# Autodesk Inventor assembly: Jonathan's Printer
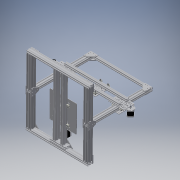
[picture p0: Inventor's stored thumbnail of the model, 180x180]
Saved by Autodesk Inventor 2016 (Build 200138000, 138)
## iProperties
Created: 2015-09-06
Part Number: Jonathan's Printer
Document SubType Name: Assembly
Designer: Solomon
Author: Solomon
## Documents named in this file (16)
- C:\Users\Solomon\Documents\Inventor\jonathan-printer\Jonathan's Printer.iam
- C:\Users\Solomon\Documents\Inventor\jonathan-printer\V Slot Part Files\Extrusions\vslot 20 x 40.ipt
- C:\Users\Solomon\Documents\Inventor\jonathan-printer\V Slot Part Files\Extrusions\vslot 20 x 20 v2.ipt
- C:\Users\Solomon\Documents\Inventor\jonathan-printer\V Slot Part Files\Brackets and Joining Plates\5 Hole 90 Degree Bracket.ipt
- C:\Users\Solomon\Documents\Inventor\jonathan-printer\V Slot Part Files\Extrusions\vslot 20 x 40 - 250mm.ipt
- C:\Users\Solomon\Documents\Inventor\jonathan-printer\V Slot Part Files\Brackets and Joining Plates\5 Hole T Joining Plate.ipt
- C:\Users\Solomon\Documents\Inventor\jonathan-printer\V Slot Part Files\Extrusions\vslot 20 x 40 - 125mm.ipt
- C:\Users\Solomon\Documents\Inventor\jonathan-printer\Z-axis Right.iam
- C:\Users\Solomon\Documents\Inventor\jonathan-printer\Z-axis Left Plate.iam
- C:\Users\Solomon\Documents\Inventor\jonathan-printer\X-carriage.iam
- C:\Users\Solomon\Documents\Inventor\jonathan-printer\y-carriage.iam
- C:\Users\Solomon\Documents\Inventor\jonathan-printer\M1173041- NEMA 17.ipt
- C:\Users\Solomon\Documents\Inventor\jonathan-printer\Imported Components\GT2_20tooth\GT2_20tooth.ipt
- C:\Users\Solomon\Documents\Inventor\jonathan-printer\V Slot Part Files\V Slot Plates\V-Slot Motor Mount Plate.ipt
- C:\Users\Solomon\Documents\Inventor\jonathan-printer\V Slot Part Files\V Slot Plates\VSlot Idler Pulley Plate.ipt
- C:\Users\Solomon\Documents\Inventor\jonathan-printer\V Slot Part Files\Pulleys Wheels Bearings\GT2 Timing Pulley.ipt
## Components (43 placed, 15 different names)
1. vslot 20 x 40:2 — Angle:1, Flush:1, Flush:3, Mate:1, Angle:2, Flush:5, Mate:6, Mate:7, Mate:8, Angle:4, Mate:16, Mate:18, Flush:47, Mate:32, Mate:33, Flush:53, Flush:54, Mate:36, Flush:57, Flush:58, Angle:16, Angle:17, Tangent:2, Mate:51
2. vslot 20 x 40:3 — Flush:2, Mate:2, Mate:3, Flush:4, Angle:3, Mate:19, Mate:20, Flush:32, Mate:29, Flush:50, Mate:31, Flush:51, Mate:38, Flush:61, Flush:62, Angle:15, Flush:75, Angle:18, Angle:20, Tangent:3
3. vslot 20 x 20 v2:1 — Angle:1, Flush:1, Flush:2, Flush:3, Mate:1, Mate:2, Mate:4, Flush:4, Flush:5, Mate:5, Flush:8, Angle:19, Angle:21, Angle:23
4. 5 Hole 90 Degree Bracket:1 — Angle:2, Mate:3, Mate:4, Flush:6, Flush:7
5. 5 Hole 90 Degree Bracket:2 — Flush:6, Flush:7, Mate:5
6. 5 Hole 90 Degree Bracket:3 — Angle:3, Mate:6, Flush:8, Mate:7, Flush:9, Flush:10
7. 5 Hole 90 Degree Bracket:4 — Flush:9, Flush:10, Mate:8
8. 5 Hole T Joining Plate:1 — Angle:4, Mate:16, Flush:25, Flush:26, Flush:27, Flush:47
9. 5 Hole T Joining Plate:2 — Flush:25, Flush:26, Flush:27, Mate:18, Flush:28, Flush:29
10. 5 Hole T Joining Plate:3 — Mate:19, Flush:28, Flush:29, Flush:30, Flush:31
11. 5 Hole T Joining Plate:4 — Mate:20, Flush:30, Flush:31, Flush:32, Mate:29
12. vslot 20 x 40 - 250mm:1 — Mate:30, Flush:48, Flush:49, Mate:31, Flush:51, Angle:5, Angle:26, Mate:56
13. vslot 20 x 40 - 250mm:2 — Mate:30, Flush:48, Flush:49, Flush:50, Angle:6, Angle:48
14. vslot 20 x 40 - 250mm:3 — Mate:33, Flush:52, Flush:53, Mate:34, Flush:64, Flush:65, Angle:29, Mate:57, Flush:83
15. vslot 20 x 40 - 250mm:4 — Mate:32, Flush:52, Mate:34, Flush:54, Flush:63, Mate:39
16. vslot 20 x 40 - 250mm:5 — Mate:35, Flush:55, Flush:56, Mate:36, Flush:58, Flush:67, Angle:8, Angle:25, Angle:32
17. vslot 20 x 40 - 250mm:6 — Mate:35, Flush:55, Flush:56, Flush:57, Mate:40, Flush:66, Mate:42, Angle:31, Mate:59, Flush:86, Angle:52
18. vslot 20 x 40 - 250mm:7 — Mate:37, Flush:59, Flush:60, Mate:38, Flush:61, Angle:9, Mate:58
19. vslot 20 x 40 - 250mm:8 — Mate:37, Flush:59, Flush:60, Flush:62, Flush:84
20. vslot 20 x 40:4 — Angle:5, Angle:6, Flush:63, Mate:39, Flush:64, Flush:65, Flush:80, Angle:27, Angle:28, Flush:81, Angle:30, Flush:82, Angle:47, Angle:57, Mate:74, Angle:59, Flush:100, Flush:102, Flush:104
21. vslot 20 x 40:5 — Mate:40, Flush:66, Flush:67, Angle:7, Mate:41, Flush:68, Flush:85, Flush:87, Angle:51, Flush:96, Mate:68, Angle:55, Mate:69
22. vslot 20 x 40 - 125mm:1 — Angle:7, Angle:8, Mate:41, Flush:68, Mate:42, Flush:69, Flush:70, Mate:43, Mate:44, Flush:71, Flush:72, Mate:67
23. vslot 20 x 40:6 — Angle:9, Flush:69, Flush:70, Mate:43, Angle:24, Tangent:5, Flush:99, Mate:75, Mate:77, Flush:103
24. vslot 20 x 40:7 — Mate:44, Flush:71, Flush:72, Mate:55, Flush:97, Mate:76, Flush:101
25. vslot 20 x 20 v2:2 — Angle:15, Flush:75, Flush:76, Mate:49, Mate:52, Flush:77
26. vslot 20 x 20 v2:3 — Flush:76, Mate:49, Mate:50, Mate:53, Tangent:4, Mate:54
27. Z-axis Right:1 [sub-assembly] — Angle:16, Angle:17, Tangent:2, Mate:50, Mate:51, Mate:52, Flush:77, Flush:78, Flush:79, Angle:22
28. Z-axis Left Plate:1 [sub-assembly] — Angle:18, Angle:19, Angle:20, Flush:78, Flush:79, Tangent:3, Mate:53
29. X-carriage:1 [sub-assembly] — Angle:21, Angle:22, Angle:23, Tangent:4, Mate:54
30. y-carriage:1 [sub-assembly] — Angle:24, Angle:25, Tangent:5, Mate:55, Angle:50
31. 5 Hole 90 Degree Bracket:5 — Angle:26, Mate:56, Flush:80, Angle:27, Angle:28, Flush:81
32. 5 Hole 90 Degree Bracket:6 — Angle:29, Angle:30, Mate:57, Flush:82, Flush:83
33. 5 Hole 90 Degree Bracket:9 — Mate:58, Flush:84, Flush:85
34. 5 Hole 90 Degree Bracket:10 — Angle:31, Angle:32, Mate:59, Flush:86, Flush:87
35. M1173041- NEMA 17:1 — Angle:47, Angle:48, Insert:1, Mate:70
36. GT2_20tooth:1 — Insert:1
37. 5 Hole 90 Degree Bracket:11 — Angle:50, Angle:51, Mate:67, Flush:96, Flush:97, Flush:98, Angle:53, Angle:54
38. 5 Hole 90 Degree Bracket:12 — Angle:52, Mate:68, Flush:98, Flush:99, Mate:73
39. V-Slot Motor Mount Plate:1 — Angle:53, Angle:54, Angle:55, Mate:69, Mate:70, Mate:73
40. VSlot Idler Pulley Plate:1 — Angle:57, Angle:58, Mate:72, Mate:74, Mate:75, Angle:60, Flush:104
41. GT2 Timing Pulley:1 — Angle:58, Mate:72
42. 5 Hole 90 Degree Bracket:13 — Angle:59, Mate:76, Flush:100, Flush:101
43. 5 Hole 90 Degree Bracket:14 — Angle:60, Mate:77, Flush:102, Flush:103
## Relationships (159: Flush 66, Mate 49, Angle 39, Tangent 4, Insert 1)
- Angle:1 (0 deg): vslot 20 x 40:2 ↔ vslot 20 x 20 v2:1
- Flush:1: vslot 20 x 40:2 ↔ vslot 20 x 20 v2:1
- Flush:2: vslot 20 x 40:3 ↔ vslot 20 x 20 v2:1
- Flush:3: vslot 20 x 40:2 ↔ vslot 20 x 20 v2:1
- Mate:1: vslot 20 x 40:2 ↔ vslot 20 x 20 v2:1
- Mate:2: vslot 20 x 40:3 ↔ vslot 20 x 20 v2:1
- Angle:2 (0 deg): vslot 20 x 40:2 ↔ 5 Hole 90 Degree Bracket:1
- Mate:3: vslot 20 x 40:3 ↔ 5 Hole 90 Degree Bracket:1
- Mate:4: vslot 20 x 20 v2:1 ↔ 5 Hole 90 Degree Bracket:1
- Flush:4: vslot 20 x 40:3 ↔ vslot 20 x 20 v2:1
- Flush:5: vslot 20 x 40:2 ↔ vslot 20 x 20 v2:1
- Flush:6: 5 Hole 90 Degree Bracket:1 ↔ 5 Hole 90 Degree Bracket:2
- Flush:7: 5 Hole 90 Degree Bracket:1 ↔ 5 Hole 90 Degree Bracket:2
- Mate:5: vslot 20 x 20 v2:1 ↔ 5 Hole 90 Degree Bracket:2
- Angle:3 (0 deg): vslot 20 x 40:3 ↔ 5 Hole 90 Degree Bracket:3
- Mate:6: vslot 20 x 40:2 ↔ 5 Hole 90 Degree Bracket:3
- Flush:8: vslot 20 x 20 v2:1 ↔ 5 Hole 90 Degree Bracket:3
- Mate:7 (6.1 mm): vslot 20 x 40:2 ↔ 5 Hole 90 Degree Bracket:3
- Flush:9: 5 Hole 90 Degree Bracket:3 ↔ 5 Hole 90 Degree Bracket:4
- Flush:10: 5 Hole 90 Degree Bracket:3 ↔ 5 Hole 90 Degree Bracket:4
- Mate:8: vslot 20 x 40:2 ↔ 5 Hole 90 Degree Bracket:4
- Angle:4 (0 deg): vslot 20 x 40:2 ↔ 5 Hole T Joining Plate:1
- Mate:16 (6.1 mm): vslot 20 x 40:2 ↔ 5 Hole T Joining Plate:1
- Flush:25: 5 Hole T Joining Plate:1 ↔ 5 Hole T Joining Plate:2
- Flush:26: 5 Hole T Joining Plate:1 ↔ 5 Hole T Joining Plate:2
- Flush:27: 5 Hole T Joining Plate:1 ↔ 5 Hole T Joining Plate:2
- Mate:18 (6.1 mm): vslot 20 x 40:2 ↔ 5 Hole T Joining Plate:2
- Mate:19 (6.1 mm): vslot 20 x 40:3 ↔ 5 Hole T Joining Plate:3
- Flush:28: 5 Hole T Joining Plate:2 ↔ 5 Hole T Joining Plate:3
- Flush:29: 5 Hole T Joining Plate:2 ↔ 5 Hole T Joining Plate:3
- Mate:20: vslot 20 x 40:3 ↔ 5 Hole T Joining Plate:4
- Flush:30: 5 Hole T Joining Plate:3 ↔ 5 Hole T Joining Plate:4
- Flush:31: 5 Hole T Joining Plate:3 ↔ 5 Hole T Joining Plate:4
- Flush:32: vslot 20 x 40:3 ↔ 5 Hole T Joining Plate:4
- Mate:29: vslot 20 x 40:3 ↔ 5 Hole T Joining Plate:4
- Flush:47 (-20 mm): vslot 20 x 40:2 ↔ 5 Hole T Joining Plate:1
- Mate:30: vslot 20 x 40 - 250mm:1 ↔ vslot 20 x 40 - 250mm:2
- Flush:48: vslot 20 x 40 - 250mm:1 ↔ vslot 20 x 40 - 250mm:2
- Flush:49: vslot 20 x 40 - 250mm:1 ↔ vslot 20 x 40 - 250mm:2
- Flush:50: vslot 20 x 40:3 ↔ vslot 20 x 40 - 250mm:2
- Mate:31: vslot 20 x 40:3 ↔ vslot 20 x 40 - 250mm:1
- Flush:51: vslot 20 x 40:3 ↔ vslot 20 x 40 - 250mm:1
- Mate:32: vslot 20 x 40:2 ↔ vslot 20 x 40 - 250mm:4
- Mate:33: vslot 20 x 40:2 ↔ vslot 20 x 40 - 250mm:3
- Flush:52: vslot 20 x 40 - 250mm:3 ↔ vslot 20 x 40 - 250mm:4
- Flush:53: vslot 20 x 40:2 ↔ vslot 20 x 40 - 250mm:3
- Mate:34: vslot 20 x 40 - 250mm:3 ↔ vslot 20 x 40 - 250mm:4
- Flush:54: vslot 20 x 40:2 ↔ vslot 20 x 40 - 250mm:4
- Mate:35: vslot 20 x 40 - 250mm:5 ↔ vslot 20 x 40 - 250mm:6
- Flush:55: vslot 20 x 40 - 250mm:5 ↔ vslot 20 x 40 - 250mm:6
- Flush:56: vslot 20 x 40 - 250mm:5 ↔ vslot 20 x 40 - 250mm:6
- Mate:36: vslot 20 x 40:2 ↔ vslot 20 x 40 - 250mm:5
- Flush:57: vslot 20 x 40:2 ↔ vslot 20 x 40 - 250mm:6
- Flush:58: vslot 20 x 40:2 ↔ vslot 20 x 40 - 250mm:5
- Mate:37: vslot 20 x 40 - 250mm:7 ↔ vslot 20 x 40 - 250mm:8
- Flush:59: vslot 20 x 40 - 250mm:7 ↔ vslot 20 x 40 - 250mm:8
- Flush:60: vslot 20 x 40 - 250mm:7 ↔ vslot 20 x 40 - 250mm:8
- Mate:38: vslot 20 x 40:3 ↔ vslot 20 x 40 - 250mm:7
- Flush:61: vslot 20 x 40:3 ↔ vslot 20 x 40 - 250mm:7
- Flush:62: vslot 20 x 40:3 ↔ vslot 20 x 40 - 250mm:8
- Angle:5 (0 deg): vslot 20 x 40 - 250mm:1 ↔ vslot 20 x 40:4
- Angle:6 (0 deg): vslot 20 x 40 - 250mm:2 ↔ vslot 20 x 40:4
- Flush:63: vslot 20 x 40 - 250mm:4 ↔ vslot 20 x 40:4
- Mate:39: vslot 20 x 40 - 250mm:4 ↔ vslot 20 x 40:4
- Flush:64: vslot 20 x 40 - 250mm:3 ↔ vslot 20 x 40:4
- Flush:65: vslot 20 x 40 - 250mm:3 ↔ vslot 20 x 40:4
- Mate:40: vslot 20 x 40 - 250mm:6 ↔ vslot 20 x 40:5
- Flush:66: vslot 20 x 40 - 250mm:6 ↔ vslot 20 x 40:5
- Flush:67: vslot 20 x 40 - 250mm:5 ↔ vslot 20 x 40:5
- Angle:7 (0 deg): vslot 20 x 40:5 ↔ vslot 20 x 40 - 125mm:1
- Angle:8 (0 deg): vslot 20 x 40 - 250mm:5 ↔ vslot 20 x 40 - 125mm:1
- Mate:41: vslot 20 x 40:5 ↔ vslot 20 x 40 - 125mm:1
- Flush:68: vslot 20 x 40:5 ↔ vslot 20 x 40 - 125mm:1
- Mate:42 (147.5 mm): vslot 20 x 40 - 250mm:6 ↔ vslot 20 x 40 - 125mm:1
- Angle:9 (0 deg): vslot 20 x 40 - 250mm:7 ↔ vslot 20 x 40:6
- Flush:69 (22.5 mm): vslot 20 x 40 - 125mm:1 ↔ vslot 20 x 40:6
- Flush:70: vslot 20 x 40 - 125mm:1 ↔ vslot 20 x 40:6
- Mate:43: vslot 20 x 40 - 125mm:1 ↔ vslot 20 x 40:6
- Mate:44: vslot 20 x 40 - 125mm:1 ↔ vslot 20 x 40:7
- Flush:71 (22.5 mm): vslot 20 x 40 - 125mm:1 ↔ vslot 20 x 40:7
- Flush:72: vslot 20 x 40 - 125mm:1 ↔ vslot 20 x 40:7
- Angle:15 (0 deg): vslot 20 x 40:3 ↔ vslot 20 x 20 v2:2
- Flush:75: vslot 20 x 40:3 ↔ vslot 20 x 20 v2:2
- Flush:76: vslot 20 x 20 v2:2 ↔ vslot 20 x 20 v2:3
- Mate:49 (40 mm): vslot 20 x 20 v2:2 ↔ vslot 20 x 20 v2:3
- Angle:16 (0 deg): vslot 20 x 40:2 ↔ Z-axis Right:1
- Angle:17 (0 deg): vslot 20 x 40:2 ↔ Z-axis Right:1
- Tangent:2 (4.5 mm): vslot 20 x 40:2 ↔ Z-axis Right:1
- Mate:50: vslot 20 x 20 v2:3 ↔ Z-axis Right:1
- Mate:51 (3 mm): vslot 20 x 40:2 ↔ Z-axis Right:1
- Mate:52: vslot 20 x 20 v2:2 ↔ Z-axis Right:1
- Flush:77 (4 mm): vslot 20 x 20 v2:2 ↔ Z-axis Right:1
- Angle:18 (0 deg): vslot 20 x 40:3 ↔ Z-axis Left Plate:1
- Angle:19 (0 deg): vslot 20 x 20 v2:1 ↔ Z-axis Left Plate:1
- Angle:20 (0 deg): vslot 20 x 40:3 ↔ Z-axis Left Plate:1
- Flush:78: Z-axis Right:1 ↔ Z-axis Left Plate:1
- Flush:79: Z-axis Right:1 ↔ Z-axis Left Plate:1
- Tangent:3 (4.5 mm): vslot 20 x 40:3 ↔ Z-axis Left Plate:1
- Mate:53: vslot 20 x 20 v2:3 ↔ Z-axis Left Plate:1
- Angle:21 (0 deg): vslot 20 x 20 v2:1 ↔ X-carriage:1
- Angle:22 (180 deg): Z-axis Right:1 ↔ X-carriage:1
- Angle:23 (0 deg): vslot 20 x 20 v2:1 ↔ X-carriage:1
- Tangent:4 (4.5 mm): vslot 20 x 20 v2:3 ↔ X-carriage:1
- Mate:54 (3 mm): vslot 20 x 20 v2:3 ↔ X-carriage:1
- Angle:24 (0 deg): vslot 20 x 40:6 ↔ y-carriage:1
- Angle:25 (0 deg): vslot 20 x 40 - 250mm:5 ↔ y-carriage:1
- Tangent:5 (4.5 mm): vslot 20 x 40:6 ↔ y-carriage:1
- Mate:55 (3 mm): vslot 20 x 40:7 ↔ y-carriage:1
- Angle:26 (0 deg): vslot 20 x 40 - 250mm:1 ↔ 5 Hole 90 Degree Bracket:5
- Mate:56: vslot 20 x 40 - 250mm:1 ↔ 5 Hole 90 Degree Bracket:5
- Flush:80: vslot 20 x 40:4 ↔ 5 Hole 90 Degree Bracket:5
- Angle:27 (0 deg): vslot 20 x 40:4 ↔ 5 Hole 90 Degree Bracket:5
- Angle:28 (0 deg): vslot 20 x 40:4 ↔ 5 Hole 90 Degree Bracket:5
- Flush:81: vslot 20 x 40:4 ↔ 5 Hole 90 Degree Bracket:5
- Angle:29 (0 deg): vslot 20 x 40 - 250mm:3 ↔ 5 Hole 90 Degree Bracket:6
- Angle:30 (180 deg): vslot 20 x 40:4 ↔ 5 Hole 90 Degree Bracket:6
- Mate:57: vslot 20 x 40 - 250mm:3 ↔ 5 Hole 90 Degree Bracket:6
- Flush:82: vslot 20 x 40:4 ↔ 5 Hole 90 Degree Bracket:6
- Flush:83: vslot 20 x 40 - 250mm:3 ↔ 5 Hole 90 Degree Bracket:6
- Mate:58: vslot 20 x 40 - 250mm:7 ↔ 5 Hole 90 Degree Bracket:9
- Flush:84: vslot 20 x 40 - 250mm:8 ↔ 5 Hole 90 Degree Bracket:9
- Flush:85: vslot 20 x 40:5 ↔ 5 Hole 90 Degree Bracket:9
- Angle:31 (0 deg): vslot 20 x 40 - 250mm:6 ↔ 5 Hole 90 Degree Bracket:10
- Angle:32 (0 deg): vslot 20 x 40 - 250mm:5 ↔ 5 Hole 90 Degree Bracket:10
- Mate:59: vslot 20 x 40 - 250mm:6 ↔ 5 Hole 90 Degree Bracket:10
- Flush:86: vslot 20 x 40 - 250mm:6 ↔ 5 Hole 90 Degree Bracket:10
- Flush:87: vslot 20 x 40:5 ↔ 5 Hole 90 Degree Bracket:10
- Angle:47 (0 deg): vslot 20 x 40:4 ↔ M1173041- NEMA 17:1
- Angle:48 (0 deg): vslot 20 x 40 - 250mm:2 ↔ M1173041- NEMA 17:1
- Insert:1 (-20 mm): M1173041- NEMA 17:1 ↔ GT2_20tooth:1
- Angle:50 (0 deg): y-carriage:1 ↔ 5 Hole 90 Degree Bracket:11
- Angle:51 (0 deg): vslot 20 x 40:5 ↔ 5 Hole 90 Degree Bracket:11
- Mate:67: vslot 20 x 40 - 125mm:1 ↔ 5 Hole 90 Degree Bracket:11
- Flush:96: vslot 20 x 40:5 ↔ 5 Hole 90 Degree Bracket:11
- Flush:97: vslot 20 x 40:7 ↔ 5 Hole 90 Degree Bracket:11
- Angle:52 (0 deg): vslot 20 x 40 - 250mm:6 ↔ 5 Hole 90 Degree Bracket:12
- Mate:68: vslot 20 x 40:5 ↔ 5 Hole 90 Degree Bracket:12
- Flush:98: 5 Hole 90 Degree Bracket:11 ↔ 5 Hole 90 Degree Bracket:12
- Flush:99 (1.5 mm): vslot 20 x 40:6 ↔ 5 Hole 90 Degree Bracket:12
- Angle:53 (0 deg): 5 Hole 90 Degree Bracket:11 ↔ V-Slot Motor Mount Plate:1
- Angle:54 (0 deg): 5 Hole 90 Degree Bracket:11 ↔ V-Slot Motor Mount Plate:1
- Angle:55 (0 deg): vslot 20 x 40:5 ↔ V-Slot Motor Mount Plate:1
- Mate:69: vslot 20 x 40:5 ↔ V-Slot Motor Mount Plate:1
- Mate:70: M1173041- NEMA 17:1 ↔ V-Slot Motor Mount Plate:1
- Angle:57 (0 deg): vslot 20 x 40:4 ↔ VSlot Idler Pulley Plate:1
- Angle:58 (180 deg): VSlot Idler Pulley Plate:1 ↔ GT2 Timing Pulley:1
- Mate:72: VSlot Idler Pulley Plate:1 ↔ GT2 Timing Pulley:1
- Mate:73 (1 mm): 5 Hole 90 Degree Bracket:12 ↔ V-Slot Motor Mount Plate:1
- Mate:74: vslot 20 x 40:4 ↔ VSlot Idler Pulley Plate:1
- Mate:75 (0.5 mm): vslot 20 x 40:6 ↔ VSlot Idler Pulley Plate:1
- Angle:59 (0 deg): vslot 20 x 40:4 ↔ 5 Hole 90 Degree Bracket:13
- Mate:76: vslot 20 x 40:7 ↔ 5 Hole 90 Degree Bracket:13
- Flush:100: vslot 20 x 40:4 ↔ 5 Hole 90 Degree Bracket:13
- Flush:101: vslot 20 x 40:7 ↔ 5 Hole 90 Degree Bracket:13
- Angle:60 (0 deg): VSlot Idler Pulley Plate:1 ↔ 5 Hole 90 Degree Bracket:14
- Mate:77: vslot 20 x 40:6 ↔ 5 Hole 90 Degree Bracket:14
- Flush:102: vslot 20 x 40:4 ↔ 5 Hole 90 Degree Bracket:14
- Flush:103: vslot 20 x 40:6 ↔ 5 Hole 90 Degree Bracket:14
- Flush:104: vslot 20 x 40:4 ↔ VSlot Idler Pulley Plate:1
